# Autodesk Inventor assembly: Cyclops^2
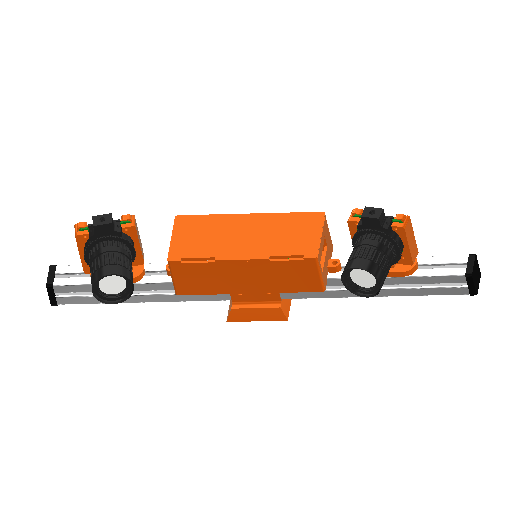
[picture p0: Inventor's stored thumbnail of the model, 512x512]
Saved by Autodesk Inventor 2025.2 (Build 292293000, 293)
## iProperties
Created: 2026-05-17
Part Number: Cyclops^2
Document SubType Name: Assembly
Designer: rolan
Author: rolan
## Documents named in this file (9)
- C:\Users\rolan\Documents\PhD\Inventor\Assembly\Cyclops^2.iam
- C:\Users\rolan\Documents\PhD\Inventor\Parts\EndCap.ipt
- C:\Users\rolan\Documents\PhD\Inventor\Parts\Strut.ipt
- C:\Users\rolan\Documents\PhD\Inventor\Parts\M12StereoPiBracket.ipt
- C:\Users\rolan\Documents\PhD\Inventor\3D Files\stereopi_v2\stereopi_v2\stereopi_v2.ipt
- C:\Users\rolan\Documents\PhD\Inventor\Parts\Tripod mount1.ipt
- C:\Users\rolan\Documents\PhD\Inventor\Parts\StereoPiBracketLidM12.ipt
- C:\Users\rolan\Documents\PhD\Inventor\Parts\CameraAngle22.5.ipt
- C:\Users\rolan\Documents\PhD\Inventor\Assembly\Camera.iam
## Components (11 placed, 8 different names)
1. Strut:1 — Mate:1, Mate:2, Mate:3, Mate:4, Mate:5, Mate:6, Mate:7, Mate:8, Flush:1, Mate:12, Mate:13, Mate:18, Mate:19, Mate:20, Flush:7, Mate:23, Mate:26
2. EndCap:1 — Mate:4, Mate:5, Mate:6
3. EndCap:2 — Mate:1, Mate:2, Mate:3
4. M12StereoPiBracket:1 — Mate:7, Mate:8, Flush:2, Mate:9, Mate:10, Mate:11, Mate:15, Mate:16, Mate:17
5. stereopi_v2:1 — Mate:9, Mate:10, Mate:11
6. Tripod mount1:1 — Mate:12, Mate:13, Mate:14
7. StereoPiBracketLidM12:1 — Mate:15, Mate:16, Mate:17
8. CameraAngle22.5:1 — Mate:18, Mate:19, Flush:6, Mate:24, Mate:25
9. CameraAngle22.5:2 — Flush:5, Mate:20, Flush:7, Mate:21, Mate:22
10. Camera:1 [sub-assembly] — Mate:21, Mate:22, Mate:23
11. Camera:2 [sub-assembly] — Mate:24, Mate:25, Mate:26
## Relationships (33: Mate 26, Flush 7)
- Mate:1: Strut:1 ↔ EndCap:2
- Mate:2: Strut:1 ↔ EndCap:2
- Mate:3: Strut:1 ↔ EndCap:2
- Mate:4: Strut:1 ↔ EndCap:1
- Mate:5: Strut:1 ↔ EndCap:1
- Mate:6: Strut:1 ↔ EndCap:1
- Mate:7: Strut:1 ↔ M12StereoPiBracket:1
- Mate:8: Strut:1 ↔ M12StereoPiBracket:1
- Flush:1 (150 mm): Strut:1
- Flush:2: M12StereoPiBracket:1
- Mate:9: M12StereoPiBracket:1 ↔ stereopi_v2:1
- Mate:10: M12StereoPiBracket:1 ↔ stereopi_v2:1
- Mate:11: M12StereoPiBracket:1 ↔ stereopi_v2:1
- Mate:12: Strut:1 ↔ Tripod mount1:1
- Mate:13: Strut:1 ↔ Tripod mount1:1
- Mate:14: Tripod mount1:1
- Mate:15: M12StereoPiBracket:1 ↔ StereoPiBracketLidM12:1
- Mate:16: M12StereoPiBracket:1 ↔ StereoPiBracketLidM12:1
- Mate:17: M12StereoPiBracket:1 ↔ StereoPiBracketLidM12:1
- Mate:18: Strut:1 ↔ CameraAngle22.5:1
- Mate:19: Strut:1 ↔ CameraAngle22.5:1
- Flush:3 (-100 mm)
- Flush:4 (100 mm)
- Flush:5: CameraAngle22.5:2
- Flush:6: CameraAngle22.5:1
- Mate:20: Strut:1 ↔ CameraAngle22.5:2
- Flush:7: Strut:1 ↔ CameraAngle22.5:2
- Mate:21: CameraAngle22.5:2 ↔ Camera:1
- Mate:22: CameraAngle22.5:2 ↔ Camera:1
- Mate:23: Strut:1 ↔ Camera:1
- Mate:24: CameraAngle22.5:1 ↔ Camera:2
- Mate:25: CameraAngle22.5:1 ↔ Camera:2
- Mate:26: Strut:1 ↔ Camera:2
